# Autodesk Inventor assembly: sugarAssembly
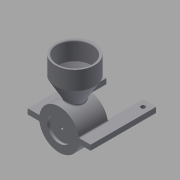
[picture p0: Inventor's stored thumbnail of the model, 180x180]
Saved by Autodesk Inventor 2017 (Build 210142000, 142)
## iProperties
Created: 2019-05-10
Part Number: sugarAssembly
Document SubType Name: Assembly
Designer: Joe Sedutto
Author: Joe Sedutto
## Documents named in this file (3)
- C:\Google Drive\Google Drive (josedutto20@sau8.org)\Classes\CRTC\Computer Engineering\CE2\CE-2-Automated-System\CAD\Subsystems\Sugar Dispensal System\sugarAssembly.iam
- C:\Google Drive\Google Drive (josedutto20@sau8.org)\Classes\CRTC\Computer Engineering\CE2\CE-2-Automated-System\CAD\Subsystems\Sugar Dispensal System\powderTurn.ipt
- C:\Google Drive\Google Drive (josedutto20@sau8.org)\Classes\CRTC\Computer Engineering\CE2\CE-2-Automated-System\CAD\Subsystems\Sugar Dispensal System\powderTurnRes.ipt
## Components (2 placed, 2 different names)
1. powderTurn:1 — Rotational:1
2. powderTurnRes:1 — Rotational:1
## Relationships (1: RevoluteJoint 1)
- Rotational:1 [RevoluteJoint]: powderTurn:1 ↔ powderTurnRes:1
